# Autodesk Inventor assembly: Zespół1
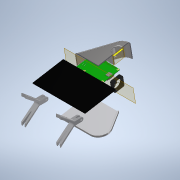
[picture p0: Inventor's stored thumbnail of the model, 180x180]
Saved by Autodesk Inventor 2020 (Build 240168000, 168)
## iProperties
Created: 2019-11-17
Part Number: Zespół1
Material: Ogólny
Document SubType Name: Assembly
Designer: macie
Author: macie
## Documents named in this file (7)
- D:\Pulpit\fotobudka\fotobudka_cad\Zespół1.iam
- D:\Pulpit\rp4\Raspberry Pi 4 Model B.ipt
- D:\Pulpit\fotobudka\fotobudka_cad\obudowa.ipt
- D:\Pulpit\fotobudka\fotobudka_cad\WIATRAK.ipt
- D:\Pulpit\fotobudka\fotobudka_cad\noga.ipt
- D:\Pulpit\fotobudka\fotobudka_cad\ekran.ipt
- D:\Pulpit\fotobudka\fotobudka_cad\klapka.ipt
## Components (7 placed, 6 different names)
1. Raspberry Pi 4 Model B:1 — Zestawiające:18, Zestawiające:19, Zestawiające:20
2. obudowa:1 — Zestawiające:3, Zestawiające:4, Zestawiające:6, Zestawiające:7, Zestawiające:12, Zestawiające:13, Kątowe:1, Zestawiające:14, Kątowe:2, Zestawiające:15, Zestawiające:16, Zestawiające:17, Równoległe:1, Równoległe:2, Zestawiające:18, Zestawiające:19, Zestawiające:20
3. WIATRAK:1 — Zestawiające:12, Zestawiające:13, Kątowe:1
4. noga:1 — Zestawiające:3, Zestawiające:4
5. noga:2 — Zestawiające:6, Zestawiające:7
6. ekran:1 — Zestawiające:14, Kątowe:2, Zestawiające:15, Zestawiające:16
7. klapka:1 — Zestawiające:17, Równoległe:1, Równoległe:2
## Relationships (17: Mate 13, Angle 2, Flush 2)
- Zestawiające:3 [Mate]: obudowa:1 ↔ noga:1
- Zestawiające:4 [Mate]: obudowa:1 ↔ noga:1
- Zestawiające:6 [Mate]: obudowa:1 ↔ noga:2
- Zestawiające:7 [Mate]: obudowa:1 ↔ noga:2
- Zestawiające:12 [Mate]: obudowa:1 ↔ WIATRAK:1
- Zestawiające:13 [Mate]: obudowa:1 ↔ WIATRAK:1
- Kątowe:1 [Angle] (0 deg): obudowa:1 ↔ WIATRAK:1
- Zestawiające:14 [Mate]: obudowa:1 ↔ ekran:1
- Kątowe:2 [Angle] (0 deg): obudowa:1 ↔ ekran:1
- Zestawiające:15 [Mate] (-2 mm): obudowa:1 ↔ ekran:1
- Zestawiające:16 [Mate] (-2 mm): obudowa:1 ↔ ekran:1
- Zestawiające:17 [Mate]: obudowa:1 ↔ klapka:1
- Równoległe:1 [Flush]: obudowa:1 ↔ klapka:1
- Równoległe:2 [Flush]: obudowa:1 ↔ klapka:1
- Zestawiające:18 [Mate]: Raspberry Pi 4 Model B:1 ↔ obudowa:1
- Zestawiające:19 [Mate]: Raspberry Pi 4 Model B:1 ↔ obudowa:1
- Zestawiające:20 [Mate]: Raspberry Pi 4 Model B:1 ↔ obudowa:1
